# Autodesk Inventor assembly: 140
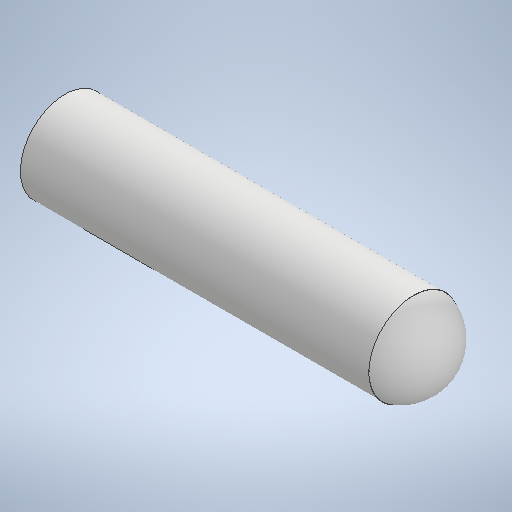
[picture p0: Inventor's stored thumbnail of the model, 512x512]
Saved by Autodesk Inventor 2025.1 (Build 291241000, 241)
## iProperties
Created: 2024-08-05
Part Number: 140
Document SubType Name: Assembly
Designer: ffogue
Author: ffogue
## Documents named in this file (3)
- C:\Projkete - Übungen\Freedom\140.iam
- C:\Projkete - Übungen\Freedom\140.ipt
- C:\Projkete - Übungen\Freedom\140 cap.ipt
## Components (2 placed, 2 different names)
1. 140:1 — Mate:1, Insert:1
2. 140 cap:1 — Mate:1, Insert:1
## Relationships (2: Mate 1, Insert 1)
- Mate:1: 140:1 ↔ 140 cap:1
- Insert:1: 140:1 ↔ 140 cap:1
